# Autodesk Inventor assembly: moto filter whel
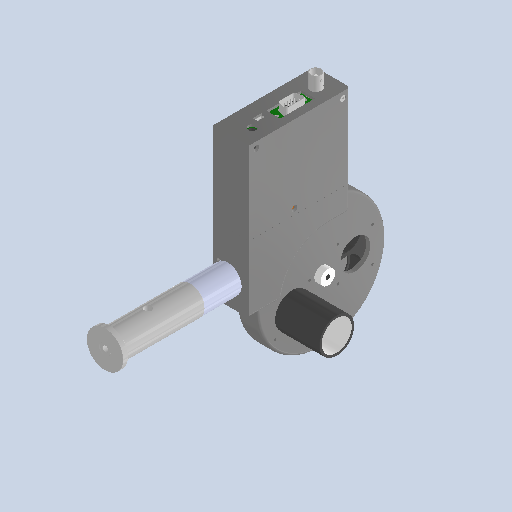
[picture p0: Inventor's stored thumbnail of the model, 512x512]
Saved by Autodesk Inventor 2026.1 (Build 301233000, 233)
## iProperties
Created: 2025-06-04
Part Number: moto filter whel
Document SubType Name: Assembly
Designer: Julian
Author: Julian
## Documents named in this file (4)
- C:\Users\user\Desktop\setup_inventor_2025\filter wheel moto\moto filter whel.iam
- C:\Users\user\Desktop\setup_inventor_2025\filter wheel moto\FW102C_partsremoved.ipt
- C:\Users\user\Desktop\setup_inventor_2025\filter wheel moto\RS3P_M.ipt
- C:\Users\user\Desktop\setup_inventor_2025\filter wheel moto\SM1L15.ipt
## Components (3 placed, 3 different names)
1. FW102C_partsremoved:1 — Passend:1, Passend:2, Passend:3, Passend:4
2. RS3P_M:1 — Passend:3, Passend:4
3. SM1L15:1 — Passend:1, Passend:2
## Relationships (4: Mate 4)
- Passend:1 [Mate]: FW102C_partsremoved:1 ↔ SM1L15:1
- Passend:2 [Mate]: FW102C_partsremoved:1 ↔ SM1L15:1
- Passend:3 [Mate]: FW102C_partsremoved:1 ↔ RS3P_M:1
- Passend:4 [Mate]: FW102C_partsremoved:1 ↔ RS3P_M:1
